# Autodesk Inventor assembly: Robot
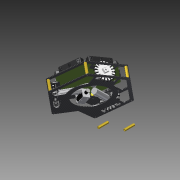
[picture p0: Inventor's stored thumbnail of the model, 180x180]
Saved by Autodesk Inventor 2015 (Build 190159000, 159)
## iProperties
Created: 2016-10-01
Part Number: Robot
Document SubType Name: Assembly
Designer: James Yelland
Author: James Yelland
## Documents named in this file (11)
- C:\Users\James Yelland\git\LJ-STAND-2017\Models\Version 2\Robot.iam
- C:\Users\James Yelland\git\LJ-STAND-2017\Models\Version 2\Bottom Plate.ipt
- C:\Users\James Yelland\git\LJ-STAND-2017\Models\Version 2\Middle Plate.ipt
- C:\Users\James Yelland\git\LJ-STAND-2017\Models\Common\Standoff 30.ipt
- C:\Users\James Yelland\git\LJ-STAND-2017\Models\Version 2\Motor Mount.ipt
- C:\Users\James Yelland\git\LJ-STAND-2017\Models\Common\Motor.ipt
- C:\Users\James Yelland\git\LJ-STAND-2017\Models\Common\Wheel.ipt
- C:\Users\James Yelland\git\LJ-STAND-2017\Models\Common\Standoff 10.ipt
- C:\Users\James Yelland\git\LJ-STAND-2017\Models\Version 2\PCB.ipt
- C:\Users\James Yelland\git\LJ-STAND-2017\Models\Version 2\TSOP Cover.ipt
- C:\Users\James Yelland\git\LJ-STAND-2017\Models\Common\Solenoid.ipt
## Components (27 placed, 10 different names)
1. Bottom Plate:1 — Mate:1, Mate:2, Mate:3, Mate:4, Mate:5, Mate:6, Mate:7, Mate:8, Mate:12, Mate:13, Mate:14, Mate:15, Mate:16, Mate:17, Mate:18, Mate:19, Mate:20
2. Middle Plate:1 — Mate:9, Mate:10, Mate:11, Mate:33, Mate:34, Mate:35, Mate:36, Mate:52
3. Standoff 30:1 — Mate:4, Mate:5
4. Standoff 30:2 — Mate:3, Mate:6, Mate:9, Mate:11
5. Standoff 30:3 — Mate:2, Mate:8
6. Standoff 30:4 — Mate:1, Mate:7, Mate:10
7. Motor Mount:1 — Mate:12, Mate:13, Mate:14, Mate:22, Mate:24, Mate:28
8. Motor Mount:2 — Mate:15, Mate:16, Mate:17, Mate:21, Mate:25, Mate:29
9. Motor Mount:3 — Mate:18, Mate:19, Mate:20, Mate:23, Mate:26, Mate:27
10. Motor:1 — Mate:22, Mate:24, Mate:28, Mate:30, Flush:3
11. Motor:2 — Mate:23, Mate:26, Mate:27, Mate:31, Flush:2
12. Motor:3 — Mate:21, Mate:25, Mate:29, Mate:32, Flush:1
13. Wheel:1 — Mate:30, Flush:3
14. Wheel:2 — Mate:31, Flush:2
15. Wheel:3 — Mate:32, Flush:1
16. Standoff 10:1 — Mate:34, Mate:35, Mate:38
17. Standoff 10:2 — Mate:33, Mate:36, Mate:37, Mate:39
18. PCB:1 — Mate:37, Mate:38, Mate:39, Flush:4, Mate:40, Mate:41, Flush:5, Mate:42, Mate:43, Flush:6, Mate:44, Mate:45, Flush:7, Flush:8, Flush:9, Mate:46, Mate:47, Mate:48, Mate:49, Mate:50, Mate:51
19. TSOP Cover:1 — Flush:4, Mate:40, Mate:41
20. TSOP Cover:2 — Flush:5, Mate:42, Mate:43
21. TSOP Cover:3 — Flush:6, Mate:44, Mate:45
22. TSOP Cover:4 — Flush:9, Mate:47, Mate:51
23. TSOP Cover:5 — Flush:8, Mate:48, Mate:49
24. TSOP Cover:6 — Flush:7, Mate:46, Mate:50
25. Solenoid:1 — Mate:52
26. Standoff 30:5
27. Standoff 30:6
## Relationships (61: Mate 52, Flush 9)
- Mate:1: Bottom Plate:1 ↔ Standoff 30:4
- Mate:2: Bottom Plate:1 ↔ Standoff 30:3
- Mate:3: Bottom Plate:1 ↔ Standoff 30:2
- Mate:4: Bottom Plate:1 ↔ Standoff 30:1
- Mate:5: Bottom Plate:1 ↔ Standoff 30:1
- Mate:6: Bottom Plate:1 ↔ Standoff 30:2
- Mate:7: Bottom Plate:1 ↔ Standoff 30:4
- Mate:8: Bottom Plate:1 ↔ Standoff 30:3
- Mate:9: Middle Plate:1 ↔ Standoff 30:2
- Mate:10: Middle Plate:1 ↔ Standoff 30:4
- Mate:11: Middle Plate:1 ↔ Standoff 30:2
- Mate:12: Bottom Plate:1 ↔ Motor Mount:1
- Mate:13: Bottom Plate:1 ↔ Motor Mount:1
- Mate:14: Bottom Plate:1 ↔ Motor Mount:1
- Mate:15: Bottom Plate:1 ↔ Motor Mount:2
- Mate:16: Bottom Plate:1 ↔ Motor Mount:2
- Mate:17: Bottom Plate:1 ↔ Motor Mount:2
- Mate:18: Bottom Plate:1 ↔ Motor Mount:3
- Mate:19: Bottom Plate:1 ↔ Motor Mount:3
- Mate:20: Bottom Plate:1 ↔ Motor Mount:3
- Mate:21: Motor Mount:2 ↔ Motor:3
- Mate:22: Motor Mount:1 ↔ Motor:1
- Mate:23: Motor Mount:3 ↔ Motor:2
- Mate:24: Motor Mount:1 ↔ Motor:1
- Mate:25: Motor Mount:2 ↔ Motor:3
- Mate:26: Motor Mount:3 ↔ Motor:2
- Mate:27: Motor Mount:3 ↔ Motor:2
- Mate:28: Motor Mount:1 ↔ Motor:1
- Mate:29: Motor Mount:2 ↔ Motor:3
- Mate:30: Motor:1 ↔ Wheel:1
- Mate:31: Motor:2 ↔ Wheel:2
- Mate:32: Motor:3 ↔ Wheel:3
- Flush:1 (-7 mm): Motor:3 ↔ Wheel:3
- Flush:2 (-7 mm): Motor:2 ↔ Wheel:2
- Flush:3 (-7 mm): Motor:1 ↔ Wheel:1
- Mate:33: Middle Plate:1 ↔ Standoff 10:2
- Mate:34: Middle Plate:1 ↔ Standoff 10:1
- Mate:35: Middle Plate:1 ↔ Standoff 10:1
- Mate:36: Middle Plate:1 ↔ Standoff 10:2
- Mate:37: Standoff 10:2 ↔ PCB:1
- Mate:38: Standoff 10:1 ↔ PCB:1
- Mate:39: Standoff 10:2 ↔ PCB:1
- Flush:4: PCB:1 ↔ TSOP Cover:1
- Mate:40: PCB:1 ↔ TSOP Cover:1
- Mate:41: PCB:1 ↔ TSOP Cover:1
- Flush:5: PCB:1 ↔ TSOP Cover:2
- Mate:42: PCB:1 ↔ TSOP Cover:2
- Mate:43: PCB:1 ↔ TSOP Cover:2
- Flush:6: PCB:1 ↔ TSOP Cover:3
- Mate:44: PCB:1 ↔ TSOP Cover:3
- Mate:45: PCB:1 ↔ TSOP Cover:3
- Flush:7: PCB:1 ↔ TSOP Cover:6
- Flush:8: PCB:1 ↔ TSOP Cover:5
- Flush:9: PCB:1 ↔ TSOP Cover:4
- Mate:46: PCB:1 ↔ TSOP Cover:6
- Mate:47: PCB:1 ↔ TSOP Cover:4
- Mate:48: PCB:1 ↔ TSOP Cover:5
- Mate:49: PCB:1 ↔ TSOP Cover:5
- Mate:50: PCB:1 ↔ TSOP Cover:6
- Mate:51: PCB:1 ↔ TSOP Cover:4
- Mate:52: Middle Plate:1 ↔ Solenoid:1
